# Autodesk Inventor assembly: Charging port
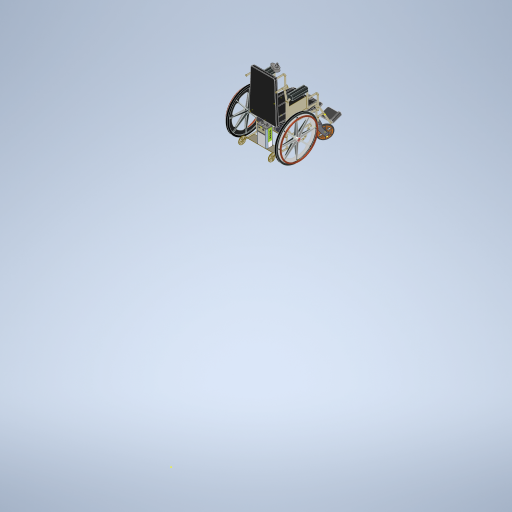
[picture p0: Inventor's stored thumbnail of the model, 512x512]
Saved by Autodesk Inventor 2023 (Build 270158000, 158)
## iProperties
Created: 2023-11-07
Part Number: Charging port
Document SubType Name: Assembly
Designer: Rahul
Author: Rahul
## Documents named in this file (4)
- C:\Users\Dell\Downloads\Charging port.iam
- C:\Users\Dell\OneDrive - iitgn.ac.in\Sem_1\ES-101\Course Project\Parts for assembly\finalproject2.ipt
- C:\Users\Dell\OneDrive - iitgn.ac.in\Sem_1\ES-101\Course Project\Parts for assembly\last.ipt
- C:\Users\Dell\OneDrive - iitgn.ac.in\Sem_1\ES-101\Final submission assembly.iam
## Components (3 placed, 3 different names)
1. finalproject2:1 — Cylindrical:1, Mate:1, Mate:2, Flush:1
2. last:1 — Cylindrical:1, Mate:1
3. Final submission assembly:1 [sub-assembly] — Mate:2, Flush:1
## Relationships (4: Mate 2, CylindricalJoint 1, Flush 1)
- Cylindrical:1: finalproject2:1 ↔ last:1
- Mate:1: finalproject2:1 ↔ last:1
- Mate:2: finalproject2:1 ↔ Final submission assembly:1
- Flush:1: finalproject2:1 ↔ Final submission assembly:1
